# Autodesk Inventor assembly: Oktokommander
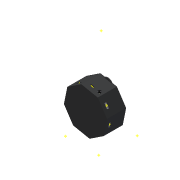
[picture p0: Inventor's stored thumbnail of the model, 180x180]
Saved by Autodesk Inventor 2018 (Build 220112000, 112)
## iProperties
Company: Fraunhofer ILT
Created: 2018-10-31
Part Number: Oktokommander
Material: geeigneten Werkstoff auswählen !
Document SubType Name: Assembly
Designer: N.Grubert
Title: =Description
Author: N.Grubert
## Documents named in this file (6)
- C:\Users\knabe\Documents\Nicole\Uni\COSIMA\CAD\Oktokommander\Oktokommander.iam
- C:\Users\knabe\Documents\Nicole\Uni\COSIMA\CAD\Oktagongehäuse\Oktagon.ipt
- C:\Users\knabe\Documents\Nicole\Uni\COSIMA\CAD\Oktagongehäuse\Oktagon_Deckel.ipt
- C:\Users\knabe\Documents\Nicole\Uni\COSIMA\CAD\Oktokommander\OktagonElektronik_Stage1.iam
- C:\Users\knabe\Documents\Nicole\Uni\COSIMA\CAD\Oktokommander\OktagonElektronik_Stage2.iam
- C:\Users\knabe\Documents\Nicole\Uni\COSIMA\CAD\Oktokommander\OktagonElektronik_Stage3.iam
## Components (5 placed, 5 different names)
1. Oktagon:1 — Passend:2, Passend:3, Passend:5, Passend:6, Passend:9, Passend:13, Passend:14, Passend:15
2. Oktagon_Deckel:1 — Passend:7, Passend:8, Passend:9, Passend:10
3. OktagonElektronik_Stage1:1 [sub-assembly] — Passend:2, Passend:3, Passend:15
4. OktagonElektronik_Stage2:1 [sub-assembly] — Passend:5, Passend:6, Passend:7, Passend:8, Passend:13
5. OktagonElektronik_Stage3:1 [sub-assembly] — Passend:10, Passend:14
## Relationships (11: Mate 11)
- Passend:2 [Mate] (1 mm): Oktagon:1 ↔ OktagonElektronik_Stage1:1
- Passend:3 [Mate] (1 mm): Oktagon:1 ↔ OktagonElektronik_Stage1:1
- Passend:5 [Mate] (1 mm): Oktagon:1 ↔ OktagonElektronik_Stage2:1
- Passend:6 [Mate] (1 mm): Oktagon:1 ↔ OktagonElektronik_Stage2:1
- Passend:7 [Mate]: Oktagon_Deckel:1 ↔ OktagonElektronik_Stage2:1
- Passend:8 [Mate]: Oktagon_Deckel:1 ↔ OktagonElektronik_Stage2:1
- Passend:9 [Mate]: Oktagon:1 ↔ Oktagon_Deckel:1
- Passend:10 [Mate]: Oktagon_Deckel:1 ↔ OktagonElektronik_Stage3:1
- Passend:13 [Mate]: Oktagon:1 ↔ OktagonElektronik_Stage2:1
- Passend:14 [Mate]: Oktagon:1 ↔ OktagonElektronik_Stage3:1
- Passend:15 [Mate]: Oktagon:1 ↔ OktagonElektronik_Stage1:1
